# Autodesk Inventor assembly: ConnectionToDart
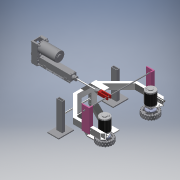
[picture p0: Inventor's stored thumbnail of the model, 180x180]
Saved by Autodesk Inventor 2017 SP1 (Build 210196100, 196)
## iProperties
Created: 2016-08-04
Part Number: ConnectionToDart
Document SubType Name: Assembly
Designer: steele
Author: steele
## Documents named in this file (8)
- D:\snobotics\CAD-Development\robSteele\SnoBotics2016\2016-05-05-ShooterPrototype\ConnectionToDart.iam
- D:\snobotics\CAD-Development\robSteele\SnoBotics2016\2016-05-05-ShooterPrototype\ShooterAssemblyForRobotV17.iam
- D:\snobotics\CAD-MfgResources\Andy-Mark\Linear Actuators\DART 6 in Actuator AM-3076a\am-3076a_DART_6_Extended.iam
- D:\snobotics\CAD-Development\robSteele\SnoBotics2016\2016-05-05-ShooterPrototype\SupportPost.ipt
- D:\snobotics\CAD-Development\robSteele\SnoBotics2016\2016-05-05-ShooterPrototype\AngleBracketAttachementForDartActuator.ipt
- D:\snobotics\CAD-Development\robSteele\SnoBotics2016\2016-05-05-ShooterPrototype\LiftAngleBracketExtensionRight.ipt
- D:\snobotics\CAD-Development\robSteele\SnoBotics2016\2016-05-05-ShooterPrototype\LiftAngleBracketExtensionLeft.ipt
- D:\snobotics\CAD-Development\robSteele\SnoBotics2016\2016-05-05-ShooterPrototype\LiftRod.ipt
## Components (8 placed, 7 different names)
1. am-3076a_DART_6_Extended:1 [sub-assembly] — Insert:6
2. ShooterAssemblyForRobotV17:1 [sub-assembly] — Insert:4, Insert:5, Mate:1, Flush:1, Flush:2, Mate:2, Flush:3, Flush:4
3. SupportPost:1 — Insert:4
4. SupportPost:2 — Insert:5
5. AngleBracketAttachementForDartActuator:2 — Insert:6, Insert:8
6. LiftAngleBracketExtensionLeft:1 — Mate:1, Flush:1, Flush:2, Insert:7
7. LiftAngleBracketExtensionRight:1 — Mate:2, Flush:3, Flush:4
8. LiftRod:1 — Insert:7, Insert:8
## Relationships (11: Insert 5, Flush 4, Mate 2)
- Insert:4: ShooterAssemblyForRobotV17:1 ↔ SupportPost:1
- Insert:5: ShooterAssemblyForRobotV17:1 ↔ SupportPost:2
- Insert:6: am-3076a_DART_6_Extended:1 ↔ AngleBracketAttachementForDartActuator:2
- Mate:1: ShooterAssemblyForRobotV17:1 ↔ LiftAngleBracketExtensionLeft:1
- Flush:1: ShooterAssemblyForRobotV17:1 ↔ LiftAngleBracketExtensionLeft:1
- Flush:2 (-203.2 mm): ShooterAssemblyForRobotV17:1 ↔ LiftAngleBracketExtensionLeft:1
- Mate:2: ShooterAssemblyForRobotV17:1 ↔ LiftAngleBracketExtensionRight:1
- Flush:3: ShooterAssemblyForRobotV17:1 ↔ LiftAngleBracketExtensionRight:1
- Flush:4 (-203.2 mm): ShooterAssemblyForRobotV17:1 ↔ LiftAngleBracketExtensionRight:1
- Insert:7 (12.7 mm): LiftAngleBracketExtensionLeft:1 ↔ LiftRod:1
- Insert:8 (-177.8 mm): AngleBracketAttachementForDartActuator:2 ↔ LiftRod:1
